# Autodesk Inventor assembly: for_bool
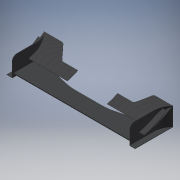
[picture p0: Inventor's stored thumbnail of the model, 180x180]
Saved by Autodesk Inventor 2018.1 (Build 221171000, 171)
## iProperties
Created: 2017-11-03
Part Number: for_bool
Material: 一般
Document SubType Name: Assembly
Designer: ku_sk
Mass: 5955.55 g
Surface Area: 13482.9 cm^2
Volume: 4164.72 cm^3
Density: 1.43 g/cm^3
Author: ku_sk
## Documents named in this file (6)
- D:\ku_sk\ドキュメント\Inventor\AeroCAD2018\CAD\Inventor\Aero Parts\F-wing\type7\parts\type7_element\for_bool.iam
- D:\ku_sk\ドキュメント\Inventor\AeroCAD2018\CAD\Inventor\Aero Parts\F-wing\type7\parts\type7_base.ipt
- D:\ku_sk\ドキュメント\Inventor\AeroCAD2018\CAD\Inventor\Aero Parts\F-wing\type7\parts\type7_end_plate.ipt
- D:\ku_sk\ドキュメント\Inventor\AeroCAD2018\CAD\Inventor\Aero Parts\F-wing\type7\parts\type7_end_plate_MIR.ipt
- D:\ku_sk\ドキュメント\Inventor\AeroCAD2018\CAD\Inventor\Aero Parts\F-wing\type7\parts\type7_element\type7_element_base_MIR.ipt
- D:\ku_sk\ドキュメント\Inventor\AeroCAD2018\CAD\Inventor\Aero Parts\F-wing\type7\parts\type7_element\type7_element_base.ipt
## Components (5 placed, 5 different names)
1. type7_base:1 — フラッシュ:1, フラッシュ:2, フラッシュ:3, メイト:1, メイト:2, フラッシュ:4, メイト:3
2. type7_end_plate:1 — メイト:1, メイト:2, フラッシュ:4, フラッシュ:5, フラッシュ:6, フラッシュ:7
3. type7_end_plate_MIR:1 — メイト:3, フラッシュ:5, フラッシュ:6, フラッシュ:8
4. type7_element_base:1 — フラッシュ:7, メイト:4, フラッシュ:9
5. type7_element_base_MIR:1 — メイト:4, フラッシュ:8, フラッシュ:9
## Relationships (13: Flush 9, Mate 4)
- フラッシュ:1 [Flush]: type7_base:1
- フラッシュ:2 [Flush]: type7_base:1
- フラッシュ:3 [Flush]: type7_base:1
- メイト:1 [Mate]: type7_base:1 ↔ type7_end_plate:1
- メイト:2 [Mate]: type7_base:1 ↔ type7_end_plate:1
- フラッシュ:4 [Flush] (30 mm): type7_base:1 ↔ type7_end_plate:1
- メイト:3 [Mate]: type7_base:1 ↔ type7_end_plate_MIR:1
- フラッシュ:5 [Flush]: type7_end_plate:1 ↔ type7_end_plate_MIR:1
- フラッシュ:6 [Flush]: type7_end_plate:1 ↔ type7_end_plate_MIR:1
- フラッシュ:7 [Flush]: type7_end_plate:1 ↔ type7_element_base:1
- メイト:4 [Mate]: type7_element_base:1 ↔ type7_element_base_MIR:1
- フラッシュ:8 [Flush]: type7_end_plate_MIR:1 ↔ type7_element_base_MIR:1
- フラッシュ:9 [Flush]: type7_element_base:1 ↔ type7_element_base_MIR:1
